# Autodesk Inventor assembly: Balcony
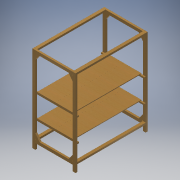
[picture p0: Inventor's stored thumbnail of the model, 180x180]
Saved by Autodesk Inventor 2019 (Build 230136000, 136)
## iProperties
Created: 2019-05-05
Part Number: Balcony
Material: Genérico
Document SubType Name: Assembly
Designer: Daniel Regner
Author: Daniel Regner
## Documents named in this file (8)
- C:\Users\Daniel Regner\Documents\GitHub\Sink-balcony\Balcony.iam
- C:\Users\Daniel Regner\Documents\GitHub\Sink-balcony\deph rip 60x80.ipt
- C:\Users\Daniel Regner\Documents\GitHub\Sink-balcony\feet rip 60x80.ipt
- C:\Users\Daniel Regner\Documents\GitHub\Sink-balcony\width rip 60x80.ipt
- C:\Users\Daniel Regner\Documents\GitHub\Sink-balcony\shelf rip 20x20.ipt
- C:\Users\Daniel Regner\Documents\GitHub\Sink-balcony\shelf.ipt
- C:\Users\Daniel Regner\Documents\GitHub\Sink-balcony\support rip.ipt
- C:\Users\Daniel Regner\Documents\GitHub\Sink-balcony\sizes.xlsx
## Components (28 placed, 6 different names)
1. deph rip 60x80:1 — Coincidência:2, Coincidência:3, Alinhamento:3, Alinhamento:4, Alinhamento:11, Coincidência:14
2. feet rip 60x80:1 — Coincidência:2, Alinhamento:4, Coincidência:7, Alinhamento:8, Coincidência:12, Alinhamento:19, Alinhamento:26, Coincidência:17, Alinhamento:29, Coincidência:24, Coincidência:26, Coincidência:41, Coincidência:47
3. width rip 60x80:1 — Coincidência:5, Alinhamento:5, Coincidência:7, Alinhamento:7, Alinhamento:25, Coincidência:32, Alinhamento:33, Coincidência:36, Alinhamento:37
4. deph rip 60x80:2 — Coincidência:1, Coincidência:4, Alinhamento:1, Alinhamento:2, Alinhamento:11, Alinhamento:12, Alinhamento:15
5. feet rip 60x80:2 — Coincidência:3, Alinhamento:3, Coincidência:8, Alinhamento:8, Alinhamento:10, Alinhamento:13, Coincidência:10, Coincidência:11, Alinhamento:18, Alinhamento:21, Alinhamento:22, Alinhamento:23, Alinhamento:27, Coincidência:42, Alinhamento:34, Coincidência:52
6. width rip 60x80:2 — Coincidência:6, Alinhamento:6, Coincidência:8, Alinhamento:7, Alinhamento:12, Alinhamento:14, Coincidência:39, Coincidência:43
7. feet rip 60x80:3 — Coincidência:1, Alinhamento:1, Coincidência:5, Alinhamento:5, Alinhamento:9, Alinhamento:20, Coincidência:16, Coincidência:22, Coincidência:27, Coincidência:33, Alinhamento:36, Coincidência:45
8. feet rip 60x80:4 — Coincidência:4, Alinhamento:2, Coincidência:6, Alinhamento:6, Alinhamento:9, Alinhamento:10, Alinhamento:13, Alinhamento:14, Coincidência:9, Alinhamento:16, Coincidência:13, Coincidência:15, Coincidência:31, Coincidência:40, Alinhamento:35, Coincidência:46
9. deph rip 60x80:3 — Coincidência:10, Alinhamento:17, Alinhamento:22, Alinhamento:28, Coincidência:18
10. width rip 60x80:3 — Coincidência:11, Alinhamento:18, Alinhamento:21, Coincidência:44, Coincidência:50, Coincidência:51, Alinhamento:38, Alinhamento:39
11. deph rip 60x80:4 — Coincidência:9, Alinhamento:15, Alinhamento:16, Alinhamento:17
12. width rip 60x80:4 — Coincidência:12, Alinhamento:19, Alinhamento:20, Coincidência:48, Coincidência:49, Alinhamento:40, Alinhamento:41
13. shelf rip 20x20:1 — Coincidência:17, Alinhamento:29, Alinhamento:31, Coincidência:19, Coincidência:21
14. shelf rip 20x20:2 — Alinhamento:27, Coincidência:15, Alinhamento:30
15. shelf rip 20x20:3 — Coincidência:16, Alinhamento:28, Coincidência:18, Alinhamento:30, Coincidência:19, Coincidência:20, Coincidência:23
16. shelf rip 20x20:4 — Coincidência:13, Alinhamento:23, Alinhamento:31, Coincidência:30
17. shelf:1 — Coincidência:26, Coincidência:29, Coincidência:30
18. shelf:2 — Coincidência:23, Coincidência:24, Coincidência:28
19. shelf:3 — Coincidência:21, Coincidência:27, Coincidência:29, Alinhamento:32
20. shelf:4 — Coincidência:20, Coincidência:22, Coincidência:28, Alinhamento:32, Coincidência:31
21. support rip:1 — Coincidência:32, Alinhamento:33, Coincidência:33, Alinhamento:36
22. support rip:4 — Coincidência:42, Coincidência:43, Alinhamento:34
23. support rip:6 — Coincidência:39, Coincidência:40, Alinhamento:35
24. support rip:8 — Coincidência:36, Coincidência:41, Alinhamento:37
25. support rip:9 — Coincidência:47, Coincidência:48, Alinhamento:41
26. support rip:10 — Coincidência:44, Coincidência:51, Alinhamento:38, Coincidência:52
27. support rip:11 — Coincidência:45, Coincidência:49, Alinhamento:40
28. support rip:12 — Coincidência:46, Coincidência:50, Alinhamento:39
## Relationships (87: Mate 47, Flush 40)
- Coincidência:1 [Mate]: deph rip 60x80:2 ↔ feet rip 60x80:3
- Coincidência:2 [Mate]: deph rip 60x80:1 ↔ feet rip 60x80:1
- Coincidência:3 [Mate]: deph rip 60x80:1 ↔ feet rip 60x80:2
- Coincidência:4 [Mate]: deph rip 60x80:2 ↔ feet rip 60x80:4
- Alinhamento:1 [Flush]: deph rip 60x80:2 ↔ feet rip 60x80:3
- Alinhamento:2 [Flush]: deph rip 60x80:2 ↔ feet rip 60x80:4
- Alinhamento:3 [Flush]: deph rip 60x80:1 ↔ feet rip 60x80:2
- Alinhamento:4 [Flush]: deph rip 60x80:1 ↔ feet rip 60x80:1
- Coincidência:5 [Mate]: width rip 60x80:1 ↔ feet rip 60x80:3
- Coincidência:6 [Mate]: width rip 60x80:2 ↔ feet rip 60x80:4
- Alinhamento:5 [Flush]: width rip 60x80:1 ↔ feet rip 60x80:3
- Alinhamento:6 [Flush]: width rip 60x80:2 ↔ feet rip 60x80:4
- Coincidência:7 [Mate]: feet rip 60x80:1 ↔ width rip 60x80:1
- Coincidência:8 [Mate]: feet rip 60x80:2 ↔ width rip 60x80:2
- Alinhamento:7 [Flush]: width rip 60x80:1 ↔ width rip 60x80:2
- Alinhamento:8 [Flush]: feet rip 60x80:1 ↔ feet rip 60x80:2
- Alinhamento:9 [Flush]: feet rip 60x80:3 ↔ feet rip 60x80:4
- Alinhamento:10 [Flush]: feet rip 60x80:2 ↔ feet rip 60x80:4
- Alinhamento:11 [Flush]: deph rip 60x80:1 ↔ deph rip 60x80:2
- Alinhamento:12 [Flush]: deph rip 60x80:2 ↔ width rip 60x80:2
- Alinhamento:13 [Flush]: feet rip 60x80:2 ↔ feet rip 60x80:4
- Alinhamento:14 [Flush] (80 mm): width rip 60x80:2 ↔ feet rip 60x80:4
- Coincidência:9 [Mate]: feet rip 60x80:4 ↔ deph rip 60x80:4
- Alinhamento:15 [Flush]: deph rip 60x80:2 ↔ deph rip 60x80:4
- Alinhamento:16 [Flush]: feet rip 60x80:4 ↔ deph rip 60x80:4
- Coincidência:10 [Mate]: feet rip 60x80:2 ↔ deph rip 60x80:3
- Alinhamento:17 [Flush]: deph rip 60x80:3 ↔ deph rip 60x80:4
- Coincidência:11 [Mate]: feet rip 60x80:2 ↔ width rip 60x80:3
- Coincidência:12 [Mate]: feet rip 60x80:1 ↔ width rip 60x80:4
- Alinhamento:18 [Flush]: feet rip 60x80:2 ↔ width rip 60x80:3
- Alinhamento:19 [Flush]: feet rip 60x80:1 ↔ width rip 60x80:4
- Alinhamento:20 [Flush]: feet rip 60x80:3 ↔ width rip 60x80:4
- Alinhamento:21 [Flush]: feet rip 60x80:2 ↔ width rip 60x80:3
- Alinhamento:22 [Flush]: feet rip 60x80:2 ↔ deph rip 60x80:3
- Coincidência:13 [Mate]: feet rip 60x80:4 ↔ shelf rip 20x20:4
- Alinhamento:23 [Flush]: feet rip 60x80:2 ↔ shelf rip 20x20:4
- Alinhamento:25 [Flush]: width rip 60x80:1
- Coincidência:14 [Mate]: deph rip 60x80:1
- Alinhamento:26 [Flush]: feet rip 60x80:1
- Alinhamento:27 [Flush]: feet rip 60x80:2 ↔ shelf rip 20x20:2
- Coincidência:15 [Mate]: feet rip 60x80:4 ↔ shelf rip 20x20:2
- Coincidência:16 [Mate]: feet rip 60x80:3 ↔ shelf rip 20x20:3
- Coincidência:17 [Mate]: feet rip 60x80:1 ↔ shelf rip 20x20:1
- Alinhamento:28 [Flush]: deph rip 60x80:3 ↔ shelf rip 20x20:3
- Alinhamento:29 [Flush]: feet rip 60x80:1 ↔ shelf rip 20x20:1
- Coincidência:18 [Mate] (500 mm): deph rip 60x80:3 ↔ shelf rip 20x20:3
- Alinhamento:30 [Flush]: shelf rip 20x20:2 ↔ shelf rip 20x20:3
- Alinhamento:31 [Flush]: shelf rip 20x20:1 ↔ shelf rip 20x20:4
- Coincidência:19 [Mate] (300 mm): shelf rip 20x20:1 ↔ shelf rip 20x20:3
- Coincidência:20 [Mate]: shelf rip 20x20:3 ↔ shelf:4
- Coincidência:21 [Mate]: shelf rip 20x20:1 ↔ shelf:3
- Coincidência:22 [Mate]: feet rip 60x80:3 ↔ shelf:4
- Coincidência:23 [Mate]: shelf rip 20x20:3 ↔ shelf:2
- Coincidência:24 [Mate]: feet rip 60x80:1 ↔ shelf:2
- Coincidência:26 [Mate]: feet rip 60x80:1 ↔ shelf:1
- Coincidência:27 [Mate]: feet rip 60x80:3 ↔ shelf:3
- Coincidência:28 [Mate]: shelf:2 ↔ shelf:4
- Coincidência:29 [Mate]: shelf:1 ↔ shelf:3
- Coincidência:30 [Mate]: shelf rip 20x20:4 ↔ shelf:1
- Alinhamento:32 [Flush]: shelf:3 ↔ shelf:4
- Coincidência:31 [Mate]: feet rip 60x80:4 ↔ shelf:4
- Coincidência:32 [Mate]: width rip 60x80:1 ↔ support rip:1
- Alinhamento:33 [Flush]: width rip 60x80:1 ↔ support rip:1
- Coincidência:33 [Mate]: feet rip 60x80:3 ↔ support rip:1
- Coincidência:36 [Mate]: width rip 60x80:1 ↔ support rip:8
- Coincidência:39 [Mate]: width rip 60x80:2 ↔ support rip:6
- Coincidência:40 [Mate]: feet rip 60x80:4 ↔ support rip:6
- Coincidência:41 [Mate]: feet rip 60x80:1 ↔ support rip:8
- Coincidência:42 [Mate]: feet rip 60x80:2 ↔ support rip:4
- Coincidência:43 [Mate]: width rip 60x80:2 ↔ support rip:4
- Alinhamento:34 [Flush]: feet rip 60x80:2 ↔ support rip:4
- Alinhamento:35 [Flush]: feet rip 60x80:4 ↔ support rip:6
- Alinhamento:36 [Flush]: feet rip 60x80:3 ↔ support rip:1
- Alinhamento:37 [Flush]: width rip 60x80:1 ↔ support rip:8
- Coincidência:44 [Mate]: width rip 60x80:3 ↔ support rip:10
- Coincidência:45 [Mate]: feet rip 60x80:3 ↔ support rip:11
- Coincidência:46 [Mate]: feet rip 60x80:4 ↔ support rip:12
- Coincidência:47 [Mate]: feet rip 60x80:1 ↔ support rip:9
- Coincidência:48 [Mate]: width rip 60x80:4 ↔ support rip:9
- Coincidência:49 [Mate]: width rip 60x80:4 ↔ support rip:11
- Coincidência:50 [Mate]: width rip 60x80:3 ↔ support rip:12
- Coincidência:51 [Mate]: width rip 60x80:3 ↔ support rip:10
- Alinhamento:38 [Flush]: width rip 60x80:3 ↔ support rip:10
- Coincidência:52 [Mate]: feet rip 60x80:2 ↔ support rip:10
- Alinhamento:39 [Flush]: width rip 60x80:3 ↔ support rip:12
- Alinhamento:40 [Flush]: width rip 60x80:4 ↔ support rip:11
- Alinhamento:41 [Flush]: width rip 60x80:4 ↔ support rip:9
## Named parameters: dist_shelf = 250 mm, RIP_H = 40 mm, RIP_L = 25 mm, HEIGHT = 1200 mm, WIDHT = 600 mm, LENGHT = 1000 mm, DIST_SINK = 500 mm, DIST_SHELF = 300 mm, FEET_H = 80 mm
